# Autodesk Inventor assembly: Hinge
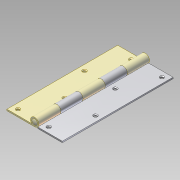
[picture p0: Inventor's stored thumbnail of the model, 180x180]
Saved by Autodesk Inventor 2012 SP2 (Build 160219200, 219)
## iProperties
Created: 2013-11-30
Part Number: Hinge
Document SubType Name: Assembly
Designer: NiveshandNisheeth
Author: NiveshandNisheeth
## Documents named in this file (4)
- C:\Users\NiveshandNisheeth\Documents\Inventor\Nivesh and Nisheeth\Hinge\Hinge.iam
- C:\Users\NiveshandNisheeth\Documents\Inventor\Nivesh and Nisheeth\Hinge\Part1.ipt
- C:\Users\NiveshandNisheeth\Documents\Inventor\Nivesh and Nisheeth\Hinge\Part2.ipt
- C:\Users\NiveshandNisheeth\Documents\Inventor\Nivesh and Nisheeth\Hinge\Centre Pin.ipt
## Components (3 placed, 3 different names)
1. Part1:1 — Mate:1, Flush:1, Drive
2. Part2:1 — Mate:1, Flush:1, Drive
3. Centre Pin:1 — Flush:2
## Relationships (4: Flush 2, Mate 1, Angle 1)
- Mate:1: Part1:1 ↔ Part2:1
- Flush:1: Part1:1 ↔ Part2:1
- Flush:2: Centre Pin:1
- Drive [Angle] (0 deg): Part1:1 ↔ Part2:1
